# Autodesk Inventor assembly: arm assembaly_MIR
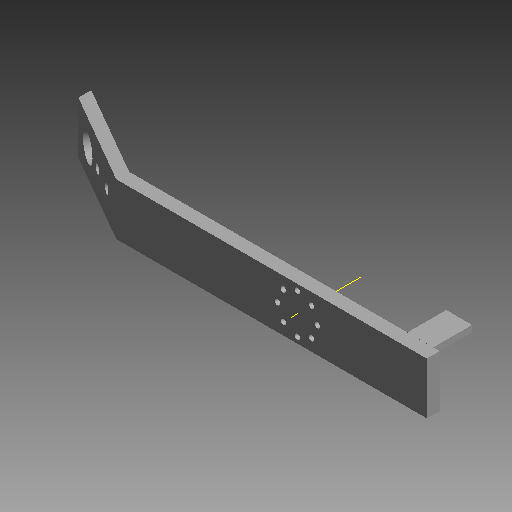
[picture p0: Inventor's stored thumbnail of the model, 512x512]
Saved by Autodesk Inventor 2019 (Build 230136000, 136)
## iProperties
Created: 2019-10-26
Part Number: arm assembaly_MIR
Document SubType Name: Assembly
Designer: Delta
Author: User
## Documents named in this file (3)
- C:\Robotics\2019-20_CAD\Collection\arm assembaly_MIR.iam
- C:\Robotics\2019-20_CAD\Collection\Wheel Arms_MIR.ipt
- C:\Robotics\2019-20_CAD\Collection\spring tab for on arm_MIR.ipt
## Components (2 placed, 2 different names)
1. Wheel Arms_MIR:1 — Flush:2, Flush:1, Mate:1
2. spring tab for on arm_MIR:1 — Flush:2, Flush:1, Mate:1
## Relationships (3: Flush 2, Mate 1)
- Flush:2 (3.175 mm): Wheel Arms_MIR:1 ↔ spring tab for on arm_MIR:1
- Flush:1: Wheel Arms_MIR:1 ↔ spring tab for on arm_MIR:1
- Mate:1: Wheel Arms_MIR:1 ↔ spring tab for on arm_MIR:1
